# Autodesk Inventor assembly: TIXEN XTY
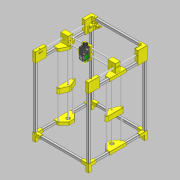
[picture p0: Inventor's stored thumbnail of the model, 180x180]
Saved by Autodesk Inventor 2020.2 (Build 242310000, 310)
## iProperties
Created: 2020-02-21
Part Number: TIXEN XTY
Document SubType Name: Assembly
Designer: TIXEN - Martin Santini
Author: TIXEN - Martin Santini
## Documents named in this file (23)
- C:\Users\TIXEN\Desktop\Core XTY\TIXEN-XTY\0.22\TIXEN XTY.iam
- C:\Users\TIXEN\Desktop\Core XTY\XTY dev\release\Ancla.ipt
- C:\Users\TIXEN\Desktop\Core XTY\XTY dev\release\Patas.ipt
- C:\Users\TIXEN\Desktop\Core XTY\XTY dev\release\Superior Back A.ipt
- C:\Users\TIXEN\Desktop\Core XTY\XTY dev\release\Superior Back B.ipt
- C:\Users\TIXEN\Desktop\Core XTY\XTY dev\release\Superior Frente A.ipt
- C:\Users\TIXEN\Desktop\Core XTY\XTY dev\release\Superior Frente B.ipt
- C:\Users\TIXEN\Desktop\Core XTY\XTY dev\release\X A.ipt
- C:\Users\TIXEN\Desktop\Core XTY\XTY dev\release\X B.ipt
- C:\Users\TIXEN\Desktop\Core XTY\XTY dev\release\Z Bottom.ipt
- C:\Users\TIXEN\Desktop\Core XTY\XTY dev\release\Z Heatbed Mount.ipt
- C:\Users\TIXEN\Desktop\Core XTY\XTY dev\release\Z TOP.ipt
- C:\Users\TIXEN\Desktop\Core XTY\XTY dev\devel\Frames\Frame Perfiles.ipt
- C:\Users\TIXEN\Desktop\Core XTY\XTY dev\devel\Frames\Varillas X.ipt
- C:\Users\TIXEN\Desktop\Core XTY\XTY dev\devel\Frames\Varillas Y.ipt
- C:\Users\TIXEN\Desktop\Core XTY\XTY dev\devel\Frames\Varillas Z.ipt
- C:\Users\TIXEN\Desktop\Core XTY\XTY dev\release\Extrusor TITAN BLTouch\B.ipt
- C:\Users\TIXEN\Desktop\Core XTY\XTY dev\release\Extrusor TITAN BLTouch\C.ipt
- C:\Users\TIXEN\Desktop\Core XTY\XTY dev\Piezas Estandar\Hot End E3D V6\E3D-HotEnd\E3D-HotEnd.iam
- C:\Users\TIXEN\Desktop\Core XTY\XTY dev\Piezas Estandar\Titan Extruder\e3d titan.iam
- C:\Users\TIXEN\Desktop\Core XTY\XTY dev\release\A.ipt
- C:\Users\TIXEN\Desktop\Core XTY\XTY dev\release\A2.ipt
- C:\Users\TIXEN\Desktop\Core XTY\XTY dev\Piezas Estandar\FAN 30X30X10.ipt
## Components (28 placed, 22 different names)
1. Frame Perfiles:1 — Mate:1, Mate:2, Mate:7, Mate:14, Mate:15, Mate:16, Mate:21, Mate:22, Mate:25, Mate:26, Mate:28, Mate:29, Mate:30, Mate:31, Mate:32, Mate:33, Mate:34, Mate:35, Mate:36, Mate:37, Mate:38, Mate:39, Mate:40, Mate:41
2. Varillas X:1 — Mate:11, Mate:19, Mate:23, Mate:44, Mate:51, Mate:52
3. Varillas Y:1 — Mate:12, Mate:13, Mate:17, Mate:18, Mate:20, Mate:24, Mate:27
4. Varillas Z:1 — Mate:3, Mate:4, Mate:5, Mate:6, Mate:8, Mate:9, Mate:10, Mate:45, Mate:46, Mate:47, Mate:48, Mate:49, Mate:50
5. E3D-HotEnd:1 [sub-assembly] — Mate:62, Mate:63
6. e3d titan:1 [sub-assembly] — Mate:62, Mate:63, Mate:69
7. FAN 30X30X10:1 — Mate:67, Mate:69, Mate:70
8. A2:1 — Mate:64, Mate:65, Mate:66, Mate:67, Mate:70
9. A:2 — Mate:64, Mate:65, Mate:66
10. B:1 — Mate:51, Mate:52, Mate:54, Flush:10, Flush:11, Mate:55, Mate:56
11. C:1 — Mate:54, Flush:10, Flush:11
12. Z Heatbed Mount:2 — Mate:47, Mate:48, Flush:6
13. Z TOP:2 — Mate:49, Mate:50, Flush:7
14. Z Bottom:2 — Mate:45, Mate:46, Flush:5
15. Ancla:1 — Mate:55, Mate:56, Angle:1
16. X A:1 — Mate:11, Mate:17, Mate:23, Mate:44
17. X B:1 — Mate:18, Mate:19
18. Z Bottom:1 — Mate:5, Mate:6, Mate:7, Mate:10, Flush:5
19. Z Heatbed Mount:1 — Mate:8, Mate:9, Flush:6
20. Z TOP:1 — Mate:1, Mate:2, Flush:4, Mate:3, Mate:4, Flush:7
21. Patas:1 — Mate:30, Mate:31, Mate:32
22. Patas:2 — Mate:39, Mate:40, Mate:41
23. Patas:3 — Mate:36, Mate:37, Mate:38
24. Patas:4 — Mate:33, Mate:34, Mate:35
25. Superior Back A:1 — Mate:12, Mate:13, Mate:14, Mate:15, Mate:16
26. Superior Back B:1 — Mate:20, Mate:21, Mate:22
27. Superior Frente A:1 — Mate:24, Mate:25, Mate:26
28. Superior Frente B:1 — Mate:27, Mate:28, Mate:29
## Relationships (77: Mate 65, Flush 11, Angle 1)
- [Flush]: Frame Perfiles:1
- [Flush]: Frame Perfiles:1
- [Flush]: Frame Perfiles:1
- Mate:1: Frame Perfiles:1 ↔ Z TOP:1
- Mate:2: Frame Perfiles:1 ↔ Z TOP:1
- Flush:4: Z TOP:1
- Mate:3: Varillas Z:1 ↔ Z TOP:1
- Mate:4: Varillas Z:1 ↔ Z TOP:1
- Mate:5: Varillas Z:1 ↔ Z Bottom:1
- Mate:6: Varillas Z:1 ↔ Z Bottom:1
- Mate:7: Frame Perfiles:1 ↔ Z Bottom:1
- Mate:8: Varillas Z:1 ↔ Z Heatbed Mount:1
- Mate:9: Varillas Z:1 ↔ Z Heatbed Mount:1
- Mate:10: Varillas Z:1 ↔ Z Bottom:1
- Mate:11: Varillas X:1 ↔ X A:1
- Mate:12: Varillas Y:1 ↔ Superior Back A:1
- Mate:13: Varillas Y:1 ↔ Superior Back A:1
- Mate:14: Frame Perfiles:1 ↔ Superior Back A:1
- Mate:15: Frame Perfiles:1 ↔ Superior Back A:1
- Mate:16: Frame Perfiles:1 ↔ Superior Back A:1
- Mate:17: Varillas Y:1 ↔ X A:1
- Mate:18: Varillas Y:1 ↔ X B:1
- Mate:19: Varillas X:1 ↔ X B:1
- Mate:20: Varillas Y:1 ↔ Superior Back B:1
- Mate:21: Frame Perfiles:1 ↔ Superior Back B:1
- Mate:22: Frame Perfiles:1 ↔ Superior Back B:1
- Mate:23: Varillas X:1 ↔ X A:1
- Mate:24: Varillas Y:1 ↔ Superior Frente A:1
- Mate:25: Frame Perfiles:1 ↔ Superior Frente A:1
- Mate:26: Frame Perfiles:1 ↔ Superior Frente A:1
- Mate:27: Varillas Y:1 ↔ Superior Frente B:1
- Mate:28: Frame Perfiles:1 ↔ Superior Frente B:1
- Mate:29: Frame Perfiles:1 ↔ Superior Frente B:1
- Mate:30: Frame Perfiles:1 ↔ Patas:1
- Mate:31: Frame Perfiles:1 ↔ Patas:1
- Mate:32: Frame Perfiles:1 ↔ Patas:1
- Mate:33: Frame Perfiles:1 ↔ Patas:4
- Mate:34: Frame Perfiles:1 ↔ Patas:4
- Mate:35: Frame Perfiles:1 ↔ Patas:4
- Mate:36: Frame Perfiles:1 ↔ Patas:3
- Mate:37: Frame Perfiles:1 ↔ Patas:3
- Mate:38: Frame Perfiles:1 ↔ Patas:3
- Mate:39: Frame Perfiles:1 ↔ Patas:2
- Mate:40: Frame Perfiles:1 ↔ Patas:2
- Mate:41: Frame Perfiles:1 ↔ Patas:2
- Mate:44: Varillas X:1 ↔ X A:1
- Mate:45: Varillas Z:1 ↔ Z Bottom:2
- Mate:46: Varillas Z:1 ↔ Z Bottom:2
- Flush:5: Z Bottom:2 ↔ Z Bottom:1
- Mate:47: Varillas Z:1 ↔ Z Heatbed Mount:2
- Mate:48: Varillas Z:1 ↔ Z Heatbed Mount:2
- Flush:6: Z Heatbed Mount:2 ↔ Z Heatbed Mount:1
- Mate:49: Varillas Z:1 ↔ Z TOP:2
- Mate:50: Varillas Z:1 ↔ Z TOP:2
- Flush:7: Z TOP:2 ↔ Z TOP:1
- Mate:51: Varillas X:1 ↔ B:1
- Mate:52: Varillas X:1 ↔ B:1
- [Flush]: A:2 ↔ B:1
- [Flush]: A:2 ↔ B:1
- Mate:54: B:1 ↔ C:1
- Flush:10: B:1 ↔ C:1
- Flush:11: B:1 ↔ C:1
- Mate:55: B:1 ↔ Ancla:1
- Mate:56: B:1 ↔ Ancla:1
- Angle:1 (0 deg): Ancla:1
- [Mate]: A:2 ↔ B:1
- [Mate]: e3d titan:1 ↔ A:2
- [Mate]: e3d titan:1 ↔ A:2
- [Mate]: e3d titan:1 ↔ A:2
- Mate:62: E3D-HotEnd:1 ↔ e3d titan:1
- Mate:63: E3D-HotEnd:1 ↔ e3d titan:1
- Mate:64: A2:1 ↔ A:2
- Mate:65: A2:1 ↔ A:2
- Mate:66: A2:1 ↔ A:2
- Mate:67: FAN 30X30X10:1 ↔ A2:1
- Mate:69 (0.5 mm): e3d titan:1 ↔ FAN 30X30X10:1
- Mate:70: FAN 30X30X10:1 ↔ A2:1
